# Autodesk Inventor assembly: Computer Case with equipment
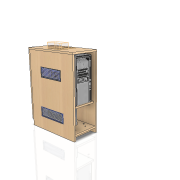
[picture p0: Inventor's stored thumbnail of the model, 180x180]
Saved by Autodesk Inventor 2024 (Build 280153000, 153)
## iProperties
Created: 2023-05-08
Part Number: Computer Case with equipment
Document SubType Name: Assembly
Designer: S. Dereškevičius
Author: S. Dereškevičius
## Documents named in this file (4)
- C:\W4INV 2024 Design\PROJECTS\Samples\Macro DEMO\7 Computer Case\Computer Case with equipment.iam
- C:\W4INV 2024 Design\PROJECTS\Samples\Macro DEMO\7 Computer Case\Computer Case.iam
- C:\W4INV 2024 Design\PROJECTS\Samples\Macro DEMO\7 Computer Case\UPS\apc_bx1400u-gr.ipt
- C:\W4INV 2024 Design\PROJECTS\Samples\Macro DEMO\7 Computer Case\Z800\HP z800.iam
## Components (3 placed, 3 different names)
1. Computer Case:1 [sub-assembly] — Flush:1, Flush:2, Flush:3, Mate:1, Mate:2
2. apc_bx1400u-gr:1 — Mate:1
3. HP z800:1 [sub-assembly] — Mate:2
## Relationships (5: Flush 3, Mate 2)
- Flush:1: Computer Case:1
- Flush:2: Computer Case:1
- Flush:3: Computer Case:1
- Mate:1: Computer Case:1 ↔ apc_bx1400u-gr:1
- Mate:2: Computer Case:1 ↔ HP z800:1
